# Autodesk Inventor assembly: GP10-100
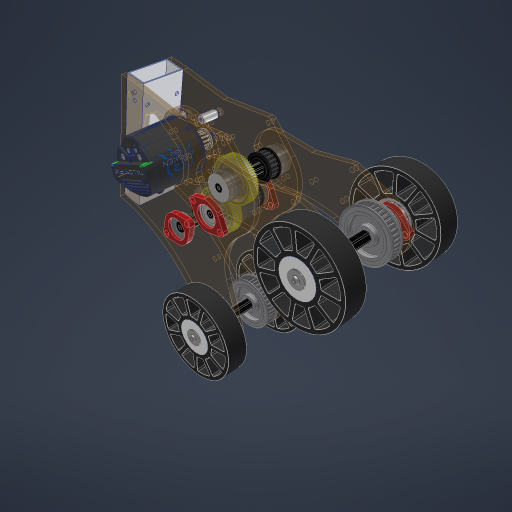
[picture p0: Inventor's stored thumbnail of the model, 512x512]
Saved by Autodesk Inventor 2023.4 (Build 274418000, 418)
## iProperties
Created: 2025-03-20
Part Number: GP10-100
Document SubType Name: Assembly
Designer: slick
Author: slick
## Documents named in this file (28)
- C:\Users\brand\OneDrive\Documents\GitHub\robotics 23\2025-ReefScape---CAD\Gripper\GP10\GP10-100.iam
- C:\Users\brand\OneDrive\Documents\GitHub\robotics 23\2025-ReefScape---CAD\Gripper\GP10\GP10-001.ipt
- C:\Users\brand\OneDrive\Documents\GitHub\robotics 23\2025-ReefScape---CAD\Gripper\GP10\GP10-002.ipt
- C:\Users\brand\OneDrive\Documents\GitHub\robotics 23\2025-ReefScape---CAD\Gripper\GP10\GP10-003.ipt
- C:\Users\brand\OneDrive\Documents\GitHub\robotics 23\2025-ReefScape---CAD\COMMON PARTS\BEARINGS\13_75mm_1_2_ThunderHex_ID_x_1_125_OD_x_0_313_WD_Flanged_Bearing_217-4006_MIR.ipt
- C:\Users\brand\OneDrive\Documents\GitHub\robotics 23\2025-ReefScape---CAD\Gripper\GP10\GP10-005.ipt
- C:\Users\brand\OneDrive\Documents\GitHub\robotics 23\2025-ReefScape---CAD\COMMON PARTS\BEARINGS\0_500_ID_x_1_125_OD_x_0_313_WD_Flanged_Bearing_217-2731.ipt
- C:\Users\brand\OneDrive\Documents\GitHub\robotics 23\2025-ReefScape---CAD\COMMON PARTS\BEARINGS\Bearing Retainer\Retainer.ipt
- C:\Users\brand\OneDrive\Documents\GitHub\robotics 23\2025-ReefScape---CAD\Gripper\GP10\GP10-007.ipt
- C:\Users\brand\OneDrive\Documents\GitHub\robotics 23\2025-ReefScape---CAD\COMMON PARTS\WHEELS\am-3480 4IN 500Hex Bore Compliant Wheel REV2 (1).iam
- C:\Users\brand\OneDrive\Documents\GitHub\robotics 23\2025-ReefScape---CAD\COMMON PARTS\BEARINGS\0_375_ID_x_1_125_OD_x_0_313_WD_Flanged_Bearing_217-2732.ipt
- C:\Users\brand\OneDrive\Documents\GitHub\robotics 23\2025-ReefScape---CAD\Gripper\GP10\GP10-008.ipt
- C:\Users\brand\OneDrive\Documents\GitHub\robotics 23\2025-ReefScape---CAD\Gripper\GP10\GP10-009.ipt
- C:\Users\brand\OneDrive\Documents\GitHub\robotics 23\2025-ReefScape---CAD\Gripper\GP10\GP10-010.ipt
- C:\Users\brand\OneDrive\Documents\GitHub\robotics 23\2025-ReefScape---CAD\Gripper\GP10\GP10-004.ipt
- C:\Users\brand\OneDrive\Documents\GitHub\robotics 23\2025-ReefScape---CAD\COMMON PARTS\MOTORS\Kracken X60WCP-0940 (1).ipt
- C:\Users\brand\OneDrive\Documents\GitHub\robotics 23\2025-ReefScape---CAD\COMMON PARTS\PULLEYS\htd\WCP-1017 (1)\WCP-1017 (1).ipt
- C:\Users\brand\OneDrive\Documents\GitHub\robotics 23\2025-ReefScape---CAD\COMMON PARTS\PULLEYS\htd\36t_x_9mm_Wide_Double_Flange_Aluminum_Pulley_HTD_5mm_1_2_Hex_Bore_217-3231.ipt
- C:\Users\brand\OneDrive\Documents\GitHub\robotics 23\2025-ReefScape---CAD\COMMON PARTS\PULLEYS\htd\18t_x_9mm_Wide_Double_Flange_Aluminum_Pulley_HTD_5mm_1_2_Hex_Bore_217-3225.ipt
- C:\Users\brand\OneDrive\Documents\GitHub\robotics 23\2025-ReefScape---CAD\Gripper\GP10\GP10-011.ipt
- C:\Users\brand\OneDrive\Documents\GitHub\robotics 23\2025-ReefScape---CAD\Gripper\GP10\GP10-012.ipt
- C:\Users\brand\OneDrive\Documents\GitHub\robotics 23\2025-ReefScape---CAD\COMMON PARTS\GEARS\32 dp gear\60t_Aluminum_Spur_Gear_32_DP_3_8_Hex_Bore_217-5863.ipt
- C:\Users\brand\OneDrive\Documents\GitHub\robotics 23\2025-ReefScape---CAD\COMMON PARTS\PULLEYS\htd\24t_x_9mm_Wide_Double_Flange_Aluminum_Pulley_HTD_5mm_1_2_Hex_Bore_217-3227.ipt
- C:\Users\brand\OneDrive\Documents\GitHub\robotics 23\2025-ReefScape---CAD\Content Center\en-US\ANSI B18.3(03)\ANSI B18.3 - 10-32 UNF - UNF - 0.125(1).ipt
- C:\Users\brand\OneDrive\Documents\GitHub\robotics 23\2025-ReefScape---CAD\Content Center\en-US\ANSI B18.3(03)\ANSI B18.3 - 10-32 UNF - UNF - 0.5(1).ipt
- C:\Users\brand\OneDrive\Documents\GitHub\robotics 23\2025-ReefScape---CAD\Content Center\en-US\ANSI B18.3(03)\ANSI B18.3 - 10-32 UNF - UNF - 0.75(1).ipt
- C:\Users\brand\OneDrive\Documents\GitHub\robotics 23\2025-ReefScape---CAD\Content Center\en-US\ANSI B18.3(03)\ANSI B18.3 - 10-32 UNF - UNF - 1(1).ipt
- C:\Users\brand\OneDrive\Documents\GitHub\robotics 23\2025-ReefScape---CAD\Content Center\en-US\ANSI B18.22.1\ANSI B18.22.1 - No. 10 - wide - Type B.ipt
## Components (67 placed, 27 different names)
1. GP10-001:1 — Mate:1, Angle:1, Mate:3, Flush:1, Mate:5, Insert:4, Insert:9, Insert:10, Insert:21, Insert:24, Insert:25, Insert:28, Insert:29, Insert:30, Insert:31, Mate:22, Mate:24, Insert:36, Insert:38, Insert:41, Insert:42, Insert:47, Insert:48, Insert:58, Insert:62, Insert:63, Insert:67, Insert:71, Insert:72, Insert:73, Insert:82
2. GP10-002:1 — Mate:1, Angle:1, Mate:3, Mate:7, Insert:3, Insert:16, Insert:17, Insert:37
3. GP10-003:1 — Flush:1, Mate:5, Mate:6, Insert:1, Insert:11, Insert:22, Insert:26, Insert:27, Insert:35, Insert:39, Insert:43, Insert:44, Insert:45, Insert:46, Mate:37
4. GP10-002:2 — Mate:6, Mate:7, Insert:2, Insert:18, Insert:19, Insert:40
5. 13_75mm_1_2_ThunderHex_ID_x_1_125_OD_x_0_313_WD_Flanged_Bearing_217-4006_MIR:1 — Insert:3, Mate:11
6. 13_75mm_1_2_ThunderHex_ID_x_1_125_OD_x_0_313_WD_Flanged_Bearing_217-4006_MIR:2 — Insert:2
7. 13_75mm_1_2_ThunderHex_ID_x_1_125_OD_x_0_313_WD_Flanged_Bearing_217-4006_MIR:3 — Insert:1
8. 13_75mm_1_2_ThunderHex_ID_x_1_125_OD_x_0_313_WD_Flanged_Bearing_217-4006_MIR:4 — Insert:4, Mate:17, Mate:45
9. GP10-005:1 — Insert:9, Insert:10, Insert:11
10. Retainer:1 — Insert:16, Insert:17
11. Retainer:2 — Insert:18, Insert:19, Mate:14
12. GP10-007:1 — Mate:11, Mate:12, Flush:3, Mate:13, Flush:4, Mate:44, Insert:49, Insert:56
13. am-3480 4IN 500Hex Bore Compliant Wheel REV2 (1):1 [sub-assembly] — Mate:12, Flush:3
14. am-3480 4IN 500Hex Bore Compliant Wheel REV2 (1):2 [sub-assembly] — Mate:13, Flush:4, Mate:14, Insert:50
15. 0_375_ID_x_1_125_OD_x_0_313_WD_Flanged_Bearing_217-2732:3 — Insert:21, Mate:16, Flush:6, Mate:42
16. 0_375_ID_x_1_125_OD_x_0_313_WD_Flanged_Bearing_217-2732:4 — Insert:22
17. GP10-008:2 — Mate:16, Flush:6, Mate:35, Mate:38, Mate:41
18. GP10-009:1 — Mate:17, Mate:18, Flush:7, Flush:8, Mate:19, Mate:43, Insert:55, Insert:57
19. am-3480 4IN 500Hex Bore Compliant Wheel REV2 (1):3 [sub-assembly] — Mate:18, Flush:7
20. am-3480 4IN 500Hex Bore Compliant Wheel REV2 (1):4 [sub-assembly] — Flush:8, Mate:19, Mate:20
21. Retainer:3 — Insert:24, Insert:25
22. Retainer:4 — Insert:26, Insert:27, Mate:20
23. GP10-010:1 — Insert:28, Insert:32
24. GP10-010:2 — Insert:29
25. GP10-010:3 — Insert:30
26. GP10-010:4 — Insert:31, Insert:33
27. GP10-004:1 — Insert:32, Insert:33, Mate:21, Insert:34
28. Kracken X60WCP-0940 (1):1 — Mate:21, Mate:22, Insert:34, Mate:23
29. WCP-1017 (1):1 — Mate:23, Mate:24
30. 36t_x_9mm_Wide_Double_Flange_Aluminum_Pulley_HTD_5mm_1_2_Hex_Bore_217-3231:1 — Mate:28, Mate:32, Mate:33
31. 18t_x_9mm_Wide_Double_Flange_Aluminum_Pulley_HTD_5mm_1_2_Hex_Bore_217-3225:1 — Mate:28, Flush:12
32. 0_500_ID_x_1_125_OD_x_0_313_WD_Flanged_Bearing_217-2731:1 — Insert:35, Mate:31, Flush:9, Mate:32
33. 0_500_ID_x_1_125_OD_x_0_313_WD_Flanged_Bearing_217-2731:2 — Insert:36, Mate:33
34. 0_375_ID_x_1_125_OD_x_0_313_WD_Flanged_Bearing_217-2732:5 — Insert:37, Mate:29
35. 0_375_ID_x_1_125_OD_x_0_313_WD_Flanged_Bearing_217-2732:6 — Insert:38, Mate:29, Mate:39
36. 0_375_ID_x_1_125_OD_x_0_313_WD_Flanged_Bearing_217-2732:7 — Insert:40, Mate:30, Mate:34, Flush:10
37. 0_375_ID_x_1_125_OD_x_0_313_WD_Flanged_Bearing_217-2732:8 — Insert:39, Mate:30
38. Retainer:5 — Insert:43, Insert:44
39. Retainer:6 — Insert:41, Insert:42
40. Retainer:7 — Insert:47, Insert:48
41. Retainer:8 — Insert:45, Insert:46
42. GP10-011:1 — Mate:31, Flush:9
43. GP10-012:1 — Mate:34, Flush:10, Mate:36, Mate:40
44. 60t_Aluminum_Spur_Gear_32_DP_3_8_Hex_Bore_217-5863:1 — Mate:36, Flush:11
45. 60t_Aluminum_Spur_Gear_32_DP_3_8_Hex_Bore_217-5863:2 — Mate:35, Flush:11, Mate:37
46. 24t_x_9mm_Wide_Double_Flange_Aluminum_Pulley_HTD_5mm_1_2_Hex_Bore_217-3227:1 — Mate:38, Flush:12
47. 18t_x_9mm_Wide_Double_Flange_Aluminum_Pulley_HTD_5mm_1_2_Hex_Bore_217-3225:2 — Mate:39, Mate:40, Flush:13
48. 18t_x_9mm_Wide_Double_Flange_Aluminum_Pulley_HTD_5mm_1_2_Hex_Bore_217-3225:3 — Mate:41, Mate:42
49. 36t_x_9mm_Wide_Double_Flange_Aluminum_Pulley_HTD_5mm_1_2_Hex_Bore_217-3231:2 — Mate:43, Mate:45
50. 36t_x_9mm_Wide_Double_Flange_Aluminum_Pulley_HTD_5mm_1_2_Hex_Bore_217-3231:3 — Mate:44, Flush:13
51. Plain Washer (Inch) No. 10 - wide - Type B:3 — Insert:49, Insert:51
52. Hexagon Socket Button Head Cap Screw - Inch No. 10-32 - 1/8:1 — Insert:50
53. Hexagon Socket Button Head Cap Screw - Inch No. 10-32 - 1/2:1 — Insert:51
54. Plain Washer (Inch) No. 10 - wide - Type B:2 — Insert:57
55. Hexagon Socket Button Head Cap Screw - Inch No. 10-32 - 1/2:2
56. Plain Washer (Inch) No. 10 - wide - Type B:4 — Insert:56
57. Hexagon Socket Button Head Cap Screw - Inch No. 10-32 - 1/2:3
58. Plain Washer (Inch) No. 10 - wide - Type B:1 — Insert:55
59. Hexagon Socket Button Head Cap Screw - Inch No. 10-32 - 1/2:4
60. Hexagon Socket Button Head Cap Screw - Inch No. 10-32 - 3/4:1 — Insert:58
61. Hexagon Socket Button Head Cap Screw - Inch No. 10-32 - 3/4:5 — Insert:62
62. Hexagon Socket Button Head Cap Screw - Inch No. 10-32 - 3/4:6 — Insert:63
63. Hexagon Socket Button Head Cap Screw - Inch No. 10-32 - 3/4:10 — Insert:67
64. Hexagon Socket Button Head Cap Screw - Inch No. 10-32 - 3/4:14 — Insert:71
65. Hexagon Socket Button Head Cap Screw - Inch No. 10-32 - 1:1 — Insert:72
66. Hexagon Socket Button Head Cap Screw - Inch No. 10-32 - 3/4:16 — Insert:73
67. Hexagon Socket Button Head Cap Screw - Inch No. 10-32 - 3/4:25 — Insert:82
## Relationships (103: Insert 55, Mate 36, Flush 11, Angle 1)
- Mate:1: GP10-001:1 ↔ GP10-002:1
- Angle:1 (0 deg): GP10-001:1 ↔ GP10-002:1
- Mate:3: GP10-001:1 ↔ GP10-002:1
- Flush:1: GP10-001:1 ↔ GP10-003:1
- Mate:5: GP10-001:1 ↔ GP10-003:1
- Mate:6: GP10-003:1 ↔ GP10-002:2
- Mate:7: GP10-002:1 ↔ GP10-002:2
- Insert:1: GP10-003:1 ↔ 13_75mm_1_2_ThunderHex_ID_x_1_125_OD_x_0_313_WD_Flanged_Bearing_217-4006_MIR:3
- Insert:2: GP10-002:2 ↔ 13_75mm_1_2_ThunderHex_ID_x_1_125_OD_x_0_313_WD_Flanged_Bearing_217-4006_MIR:2
- Insert:3: GP10-002:1 ↔ 13_75mm_1_2_ThunderHex_ID_x_1_125_OD_x_0_313_WD_Flanged_Bearing_217-4006_MIR:1
- Insert:4: GP10-001:1 ↔ 13_75mm_1_2_ThunderHex_ID_x_1_125_OD_x_0_313_WD_Flanged_Bearing_217-4006_MIR:4
- Insert:9: GP10-001:1 ↔ GP10-005:1
- Insert:10: GP10-001:1 ↔ GP10-005:1
- Insert:11: GP10-003:1 ↔ GP10-005:1
- Insert:16: GP10-002:1 ↔ Retainer:1
- Insert:17: GP10-002:1 ↔ Retainer:1
- Insert:18: GP10-002:2 ↔ Retainer:2
- Insert:19: GP10-002:2 ↔ Retainer:2
- Mate:11: 13_75mm_1_2_ThunderHex_ID_x_1_125_OD_x_0_313_WD_Flanged_Bearing_217-4006_MIR:1 ↔ GP10-007:1
- Mate:12: GP10-007:1 ↔ am-3480 4IN 500Hex Bore Compliant Wheel REV2 (1):1
- Flush:3: GP10-007:1 ↔ am-3480 4IN 500Hex Bore Compliant Wheel REV2 (1):1
- Mate:13: GP10-007:1 ↔ am-3480 4IN 500Hex Bore Compliant Wheel REV2 (1):2
- Flush:4: GP10-007:1 ↔ am-3480 4IN 500Hex Bore Compliant Wheel REV2 (1):2
- Mate:14 (3.175 mm): Retainer:2 ↔ am-3480 4IN 500Hex Bore Compliant Wheel REV2 (1):2
- Insert:21: GP10-001:1 ↔ 0_375_ID_x_1_125_OD_x_0_313_WD_Flanged_Bearing_217-2732:3
- Insert:22: GP10-003:1 ↔ 0_375_ID_x_1_125_OD_x_0_313_WD_Flanged_Bearing_217-2732:4
- Mate:16: 0_375_ID_x_1_125_OD_x_0_313_WD_Flanged_Bearing_217-2732:3 ↔ GP10-008:2
- Flush:6: 0_375_ID_x_1_125_OD_x_0_313_WD_Flanged_Bearing_217-2732:3 ↔ GP10-008:2
- Mate:17: 13_75mm_1_2_ThunderHex_ID_x_1_125_OD_x_0_313_WD_Flanged_Bearing_217-4006_MIR:4 ↔ GP10-009:1
- Mate:18: GP10-009:1 ↔ am-3480 4IN 500Hex Bore Compliant Wheel REV2 (1):3
- Flush:7: GP10-009:1 ↔ am-3480 4IN 500Hex Bore Compliant Wheel REV2 (1):3
- Flush:8: GP10-009:1 ↔ am-3480 4IN 500Hex Bore Compliant Wheel REV2 (1):4
- Mate:19: GP10-009:1 ↔ am-3480 4IN 500Hex Bore Compliant Wheel REV2 (1):4
- Insert:24: GP10-001:1 ↔ Retainer:3
- Insert:25: GP10-001:1 ↔ Retainer:3
- Insert:26: GP10-003:1 ↔ Retainer:4
- Insert:27: GP10-003:1 ↔ Retainer:4
- Mate:20 (3.175 mm): am-3480 4IN 500Hex Bore Compliant Wheel REV2 (1):4 ↔ Retainer:4
- Insert:28: GP10-001:1 ↔ GP10-010:1
- Insert:29: GP10-001:1 ↔ GP10-010:2
- Insert:30: GP10-001:1 ↔ GP10-010:3
- Insert:31: GP10-001:1 ↔ GP10-010:4
- Insert:32: GP10-010:1 ↔ GP10-004:1
- Insert:33: GP10-010:4 ↔ GP10-004:1
- Mate:21: GP10-004:1 ↔ Kracken X60WCP-0940 (1):1
- Mate:22: GP10-001:1 ↔ Kracken X60WCP-0940 (1):1
- Insert:34: GP10-004:1 ↔ Kracken X60WCP-0940 (1):1
- Mate:23: Kracken X60WCP-0940 (1):1 ↔ WCP-1017 (1):1
- Mate:24: GP10-001:1 ↔ WCP-1017 (1):1
- Mate:28: 36t_x_9mm_Wide_Double_Flange_Aluminum_Pulley_HTD_5mm_1_2_Hex_Bore_217-3231:1 ↔ 18t_x_9mm_Wide_Double_Flange_Aluminum_Pulley_HTD_5mm_1_2_Hex_Bore_217-3225:1
- Insert:35: GP10-003:1 ↔ 0_500_ID_x_1_125_OD_x_0_313_WD_Flanged_Bearing_217-2731:1
- Insert:36: GP10-001:1 ↔ 0_500_ID_x_1_125_OD_x_0_313_WD_Flanged_Bearing_217-2731:2
- Insert:37: GP10-002:1 ↔ 0_375_ID_x_1_125_OD_x_0_313_WD_Flanged_Bearing_217-2732:5
- Insert:38: GP10-001:1 ↔ 0_375_ID_x_1_125_OD_x_0_313_WD_Flanged_Bearing_217-2732:6
- Insert:39: GP10-003:1 ↔ 0_375_ID_x_1_125_OD_x_0_313_WD_Flanged_Bearing_217-2732:8
- Insert:40: GP10-002:2 ↔ 0_375_ID_x_1_125_OD_x_0_313_WD_Flanged_Bearing_217-2732:7
- Mate:29: 0_375_ID_x_1_125_OD_x_0_313_WD_Flanged_Bearing_217-2732:5 ↔ 0_375_ID_x_1_125_OD_x_0_313_WD_Flanged_Bearing_217-2732:6
- Mate:30: 0_375_ID_x_1_125_OD_x_0_313_WD_Flanged_Bearing_217-2732:7 ↔ 0_375_ID_x_1_125_OD_x_0_313_WD_Flanged_Bearing_217-2732:8
- Insert:41: GP10-001:1 ↔ Retainer:6
- Insert:42: GP10-001:1 ↔ Retainer:6
- Insert:43: GP10-003:1 ↔ Retainer:5
- Insert:44: GP10-003:1 ↔ Retainer:5
- Insert:45: GP10-003:1 ↔ Retainer:8
- Insert:46: GP10-003:1 ↔ Retainer:8
- Insert:47: GP10-001:1 ↔ Retainer:7
- Insert:48: GP10-001:1 ↔ Retainer:7
- Mate:31: 0_500_ID_x_1_125_OD_x_0_313_WD_Flanged_Bearing_217-2731:1 ↔ GP10-011:1
- Flush:9: 0_500_ID_x_1_125_OD_x_0_313_WD_Flanged_Bearing_217-2731:1 ↔ GP10-011:1
- Mate:32: 36t_x_9mm_Wide_Double_Flange_Aluminum_Pulley_HTD_5mm_1_2_Hex_Bore_217-3231:1 ↔ 0_500_ID_x_1_125_OD_x_0_313_WD_Flanged_Bearing_217-2731:1
- Mate:33: 36t_x_9mm_Wide_Double_Flange_Aluminum_Pulley_HTD_5mm_1_2_Hex_Bore_217-3231:1 ↔ 0_500_ID_x_1_125_OD_x_0_313_WD_Flanged_Bearing_217-2731:2
- Mate:34: 0_375_ID_x_1_125_OD_x_0_313_WD_Flanged_Bearing_217-2732:7 ↔ GP10-012:1
- Flush:10: 0_375_ID_x_1_125_OD_x_0_313_WD_Flanged_Bearing_217-2732:7 ↔ GP10-012:1
- Mate:35: GP10-008:2 ↔ 60t_Aluminum_Spur_Gear_32_DP_3_8_Hex_Bore_217-5863:2
- Mate:36: GP10-012:1 ↔ 60t_Aluminum_Spur_Gear_32_DP_3_8_Hex_Bore_217-5863:1
- Flush:11: 60t_Aluminum_Spur_Gear_32_DP_3_8_Hex_Bore_217-5863:1 ↔ 60t_Aluminum_Spur_Gear_32_DP_3_8_Hex_Bore_217-5863:2
- Mate:37: GP10-003:1 ↔ 60t_Aluminum_Spur_Gear_32_DP_3_8_Hex_Bore_217-5863:2
- Mate:38: GP10-008:2 ↔ 24t_x_9mm_Wide_Double_Flange_Aluminum_Pulley_HTD_5mm_1_2_Hex_Bore_217-3227:1
- Flush:12: 18t_x_9mm_Wide_Double_Flange_Aluminum_Pulley_HTD_5mm_1_2_Hex_Bore_217-3225:1 ↔ 24t_x_9mm_Wide_Double_Flange_Aluminum_Pulley_HTD_5mm_1_2_Hex_Bore_217-3227:1
- Mate:39: 0_375_ID_x_1_125_OD_x_0_313_WD_Flanged_Bearing_217-2732:6 ↔ 18t_x_9mm_Wide_Double_Flange_Aluminum_Pulley_HTD_5mm_1_2_Hex_Bore_217-3225:2
- Mate:40: GP10-012:1 ↔ 18t_x_9mm_Wide_Double_Flange_Aluminum_Pulley_HTD_5mm_1_2_Hex_Bore_217-3225:2
- Mate:41: GP10-008:2 ↔ 18t_x_9mm_Wide_Double_Flange_Aluminum_Pulley_HTD_5mm_1_2_Hex_Bore_217-3225:3
- Mate:42: 0_375_ID_x_1_125_OD_x_0_313_WD_Flanged_Bearing_217-2732:3 ↔ 18t_x_9mm_Wide_Double_Flange_Aluminum_Pulley_HTD_5mm_1_2_Hex_Bore_217-3225:3
- Mate:43: GP10-009:1 ↔ 36t_x_9mm_Wide_Double_Flange_Aluminum_Pulley_HTD_5mm_1_2_Hex_Bore_217-3231:2
- Mate:44: GP10-007:1 ↔ 36t_x_9mm_Wide_Double_Flange_Aluminum_Pulley_HTD_5mm_1_2_Hex_Bore_217-3231:3
- Mate:45: 13_75mm_1_2_ThunderHex_ID_x_1_125_OD_x_0_313_WD_Flanged_Bearing_217-4006_MIR:4 ↔ 36t_x_9mm_Wide_Double_Flange_Aluminum_Pulley_HTD_5mm_1_2_Hex_Bore_217-3231:2
- Flush:13: 18t_x_9mm_Wide_Double_Flange_Aluminum_Pulley_HTD_5mm_1_2_Hex_Bore_217-3225:2 ↔ 36t_x_9mm_Wide_Double_Flange_Aluminum_Pulley_HTD_5mm_1_2_Hex_Bore_217-3231:3
- Insert:49: GP10-007:1 ↔ Plain Washer (Inch) No. 10 - wide - Type B:3
- Insert:50: am-3480 4IN 500Hex Bore Compliant Wheel REV2 (1):2 ↔ Hexagon Socket Button Head Cap Screw - Inch No. 10-32 - 1/8:1
- Insert:51: Plain Washer (Inch) No. 10 - wide - Type B:3 ↔ Hexagon Socket Button Head Cap Screw - Inch No. 10-32 - 1/2:1
- [Insert]: Plain Washer (Inch) No. 10 - wide - Type B:2 ↔ Hexagon Socket Button Head Cap Screw - Inch No. 10-32 - 1/2:2
- [Insert]: Plain Washer (Inch) No. 10 - wide - Type B:4 ↔ Hexagon Socket Button Head Cap Screw - Inch No. 10-32 - 1/2:3
- [Insert]: Plain Washer (Inch) No. 10 - wide - Type B:1 ↔ Hexagon Socket Button Head Cap Screw - Inch No. 10-32 - 1/2:4
- Insert:55: GP10-009:1 ↔ Plain Washer (Inch) No. 10 - wide - Type B:1
- Insert:56: GP10-007:1 ↔ Plain Washer (Inch) No. 10 - wide - Type B:4
- Insert:57: GP10-009:1 ↔ Plain Washer (Inch) No. 10 - wide - Type B:2
- Insert:58: GP10-001:1 ↔ Hexagon Socket Button Head Cap Screw - Inch No. 10-32 - 3/4:1
- Insert:62: GP10-001:1 ↔ Hexagon Socket Button Head Cap Screw - Inch No. 10-32 - 3/4:5
- Insert:63: GP10-001:1 ↔ Hexagon Socket Button Head Cap Screw - Inch No. 10-32 - 3/4:6
- Insert:67: GP10-001:1 ↔ Hexagon Socket Button Head Cap Screw - Inch No. 10-32 - 3/4:10
- Insert:71: GP10-001:1 ↔ Hexagon Socket Button Head Cap Screw - Inch No. 10-32 - 3/4:14
- Insert:72: GP10-001:1 ↔ Hexagon Socket Button Head Cap Screw - Inch No. 10-32 - 1:1
- Insert:73: GP10-001:1 ↔ Hexagon Socket Button Head Cap Screw - Inch No. 10-32 - 3/4:16
- Insert:82: GP10-001:1 ↔ Hexagon Socket Button Head Cap Screw - Inch No. 10-32 - 3/4:25
## Named parameters: d133_d130 = 0 mm, d134_d131 = 0 mm, d135_d132 = 0 mm, d136_d130 = 0 mm, d137_d131 = 0 mm, d138_d132 = 0 mm, d139_d130 = 0 mm, d140_d131 = 0 mm, d141_d132 = 0 mm
